# Autodesk Inventor assembly: LeftDriveTrainMecanum2017-18
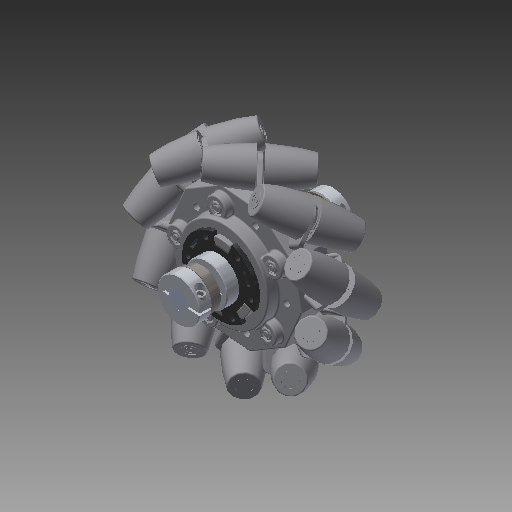
[picture p0: Inventor's stored thumbnail of the model, 512x512]
Saved by Autodesk Inventor 2017 (Build 210142000, 142)
## iProperties
Created: 2017-09-16
Part Number: LeftDriveTrainMecanum2017-18
Document SubType Name: Assembly
Designer: User
Author: User
## Documents named in this file (7)
- C:\Robotics\CAD\2017-18_CAD\LeftDriveTrainMecanum2017-18.iam
- C:\Robotics\CAD\COTSParts\Vex\HexBearings.5inchBore217-3875-STEP-20140818\HexBearings.5inchBore217-3875-STEP-20140818.ipt
- C:\Robotics\CAD\COTSParts\Vex\HexAxle.5inchOD217-3309-STEP\HexAxle.5inchOD18inchLength217-3309-STEP.ipt
- C:\Robotics\CAD\COTSParts\Vex\CollarClamp.5\am-1238+Collar+Clamp,+0.5''+Hex+Bore,+Aluminum.iam
- C:\Robotics\CAD\COTSParts\Vex\6inchMecanumLeft217-2799-STEP\6inchMecanumLeft217-2799.20121203.iam
- C:\Robotics\CAD\COTSParts\Vex\VersaHub.5inchBore217-4009-STEP-20140807\VersaHub.5inchBore217-4009-STEP-20140807.ipt
- C:\Robotics\CAD\COTSParts\Vex\HexSprocket.5inchBore\HexSprocket18t.5inchBore217-3488-STEP\HexSprocket18t.5inchBore217-3488-STEP.ipt
## Components (11 placed, 6 different names)
1. HexBearings.5inchBore217-3875-STEP-20140818:2 — Mate:5, Mate:6, Mate:8
2. HexAxle.5inchOD18inchLength217-3309-STEP:1 — Mate:5, Mate:6, Mate:7, Mate:9, Flush:1, Mate:13, Mate:14, Mate:16, Mate:17, Mate:19, Mate:20, Mate:25, Mate:26, Mate:31, Mate:32, Mate:33
3. am-1238+Collar+Clamp,+0.5''+Hex+Bore,+Aluminum:1 [sub-assembly] — Mate:7, Mate:8, Mate:9, Flush:1
4. 6inchMecanumLeft217-2799.20121203:1 [sub-assembly] — Insert:1, Mate:10, Insert:2, Mate:11
5. VersaHub.5inchBore217-4009-STEP-20140807:1 — Insert:2, Mate:11, Mate:15
6. VersaHub.5inchBore217-4009-STEP-20140807:2 — Insert:1, Mate:10, Mate:16, Mate:17, Mate:18
7. am-1238+Collar+Clamp,+0.5''+Hex+Bore,+Aluminum:2 [sub-assembly] — Mate:18, Mate:19, Mate:20
8. am-1238+Collar+Clamp,+0.5''+Hex+Bore,+Aluminum:3 [sub-assembly] — Mate:13, Mate:14, Mate:15
9. HexSprocket18t.5inchBore217-3488-STEP:1 — Mate:25, Mate:26, Mate:36
10. HexBearings.5inchBore217-3875-STEP-20140818:3 — Mate:30, Mate:33, Mate:36
11. am-1238+Collar+Clamp,+0.5''+Hex+Bore,+Aluminum:4 [sub-assembly] — Mate:30, Mate:31, Mate:32
## Relationships (25: Mate 22, Insert 2, Flush 1)
- Mate:5: HexBearings.5inchBore217-3875-STEP-20140818:2 ↔ HexAxle.5inchOD18inchLength217-3309-STEP:1
- Mate:6: HexBearings.5inchBore217-3875-STEP-20140818:2 ↔ HexAxle.5inchOD18inchLength217-3309-STEP:1
- Mate:7: HexAxle.5inchOD18inchLength217-3309-STEP:1 ↔ am-1238+Collar+Clamp,+0.5''+Hex+Bore,+Aluminum:1
- Mate:8: HexBearings.5inchBore217-3875-STEP-20140818:2 ↔ am-1238+Collar+Clamp,+0.5''+Hex+Bore,+Aluminum:1
- Mate:9: HexAxle.5inchOD18inchLength217-3309-STEP:1 ↔ am-1238+Collar+Clamp,+0.5''+Hex+Bore,+Aluminum:1
- Flush:1: HexAxle.5inchOD18inchLength217-3309-STEP:1 ↔ am-1238+Collar+Clamp,+0.5''+Hex+Bore,+Aluminum:1
- Insert:1: 6inchMecanumLeft217-2799.20121203:1 ↔ VersaHub.5inchBore217-4009-STEP-20140807:2
- Mate:10: 6inchMecanumLeft217-2799.20121203:1 ↔ VersaHub.5inchBore217-4009-STEP-20140807:2
- Insert:2: 6inchMecanumLeft217-2799.20121203:1 ↔ VersaHub.5inchBore217-4009-STEP-20140807:1
- Mate:11: 6inchMecanumLeft217-2799.20121203:1 ↔ VersaHub.5inchBore217-4009-STEP-20140807:1
- Mate:13: HexAxle.5inchOD18inchLength217-3309-STEP:1 ↔ am-1238+Collar+Clamp,+0.5''+Hex+Bore,+Aluminum:3
- Mate:14: HexAxle.5inchOD18inchLength217-3309-STEP:1 ↔ am-1238+Collar+Clamp,+0.5''+Hex+Bore,+Aluminum:3
- Mate:15: VersaHub.5inchBore217-4009-STEP-20140807:1 ↔ am-1238+Collar+Clamp,+0.5''+Hex+Bore,+Aluminum:3
- Mate:16: HexAxle.5inchOD18inchLength217-3309-STEP:1 ↔ VersaHub.5inchBore217-4009-STEP-20140807:2
- Mate:17: HexAxle.5inchOD18inchLength217-3309-STEP:1 ↔ VersaHub.5inchBore217-4009-STEP-20140807:2
- Mate:18: VersaHub.5inchBore217-4009-STEP-20140807:2 ↔ am-1238+Collar+Clamp,+0.5''+Hex+Bore,+Aluminum:2
- Mate:19: HexAxle.5inchOD18inchLength217-3309-STEP:1 ↔ am-1238+Collar+Clamp,+0.5''+Hex+Bore,+Aluminum:2
- Mate:20: HexAxle.5inchOD18inchLength217-3309-STEP:1 ↔ am-1238+Collar+Clamp,+0.5''+Hex+Bore,+Aluminum:2
- Mate:25: HexAxle.5inchOD18inchLength217-3309-STEP:1 ↔ HexSprocket18t.5inchBore217-3488-STEP:1
- Mate:26: HexAxle.5inchOD18inchLength217-3309-STEP:1 ↔ HexSprocket18t.5inchBore217-3488-STEP:1
- Mate:30: HexBearings.5inchBore217-3875-STEP-20140818:3 ↔ am-1238+Collar+Clamp,+0.5''+Hex+Bore,+Aluminum:4
- Mate:31: HexAxle.5inchOD18inchLength217-3309-STEP:1 ↔ am-1238+Collar+Clamp,+0.5''+Hex+Bore,+Aluminum:4
- Mate:32: HexAxle.5inchOD18inchLength217-3309-STEP:1 ↔ am-1238+Collar+Clamp,+0.5''+Hex+Bore,+Aluminum:4
- Mate:33: HexAxle.5inchOD18inchLength217-3309-STEP:1 ↔ HexBearings.5inchBore217-3875-STEP-20140818:3
- Mate:36: HexSprocket18t.5inchBore217-3488-STEP:1 ↔ HexBearings.5inchBore217-3875-STEP-20140818:3
